# Autodesk Inventor assembly: x_active
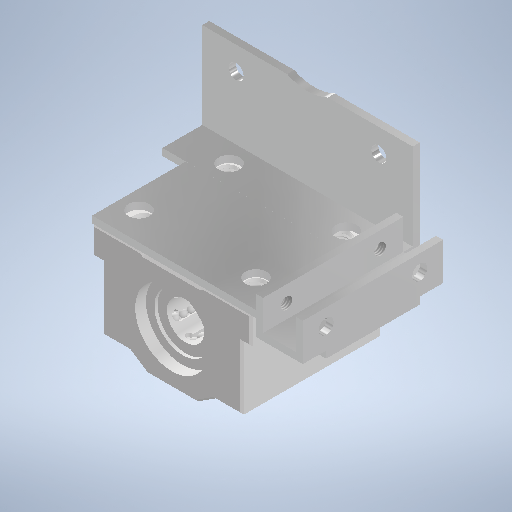
[picture p0: Inventor's stored thumbnail of the model, 512x512]
Saved by Autodesk Inventor 2025 (Build 290162000, 162)
## iProperties
Created: 2024-04-25
Part Number: x_active
Document SubType Name: Assembly
Designer: rader
Author: rader
## Documents named in this file (5)
- C:\Users\rader\Documents\rp\x_active.iam
- C:\Users\rader\Documents\rp\y_bearing.ipt
- C:\Users\rader\Documents\rp\y_anchor_holder.ipt
- C:\Users\rader\Documents\rp\x_bracket_stepper.ipt
- C:\Users\rader\Documents\rp\y_belt_anchor.ipt
## Components (4 placed, 4 different names)
1. y_bearing:1 — Proti sobě:1, Stejný směr:1, Stejný směr:2, Proti sobě:2, Stejný směr:3, Stejný směr:4, Proti sobě:3, Stejný směr:5
2. x_bracket_stepper:1 — Proti sobě:2, Stejný směr:3, Stejný směr:4, Proti sobě:4
3. y_anchor_holder:1 — Proti sobě:3, Proti sobě:4, Stejný směr:5, Vložit:1, Stejný směr:6
4. y_belt_anchor:1 — Vložit:1, Stejný směr:6
## Relationships (11: Flush 6, Mate 4, Insert 1)
- Proti sobě:1 [Mate]: y_bearing:1
- Stejný směr:1 [Flush]: y_bearing:1
- Stejný směr:2 [Flush]: y_bearing:1
- Proti sobě:2 [Mate]: y_bearing:1 ↔ x_bracket_stepper:1
- Stejný směr:3 [Flush]: y_bearing:1 ↔ x_bracket_stepper:1
- Stejný směr:4 [Flush] (-6 mm): y_bearing:1 ↔ x_bracket_stepper:1
- Proti sobě:3 [Mate]: y_bearing:1 ↔ y_anchor_holder:1
- Proti sobě:4 [Mate]: x_bracket_stepper:1 ↔ y_anchor_holder:1
- Stejný směr:5 [Flush]: y_bearing:1 ↔ y_anchor_holder:1
- Vložit:1 [Insert]: y_anchor_holder:1 ↔ y_belt_anchor:1
- Stejný směr:6 [Flush]: y_anchor_holder:1 ↔ y_belt_anchor:1
